# Autodesk Inventor assembly: wheel_kit
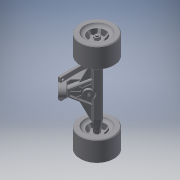
[picture p0: Inventor's stored thumbnail of the model, 180x180]
Saved by Autodesk Inventor 2017 SP1 (Build 210196100, 196)
## iProperties
Part Number: wheel_kit
Material: 一般
Document SubType Name: Assembly
Designer: gisen
Author: gisen
## Documents named in this file (5)
- C:\Users\gisen\Documents\myElectricSk8\CAD\wheel_kit.iam
- C:\Users\gisen\Documents\myElectricSk8\CAD\shaft.ipt
- C:\Users\gisen\Documents\myElectricSk8\CAD\wheel.ipt
- C:\Users\gisen\Documents\myElectricSk8\CAD\nut.ipt
- C:\Users\gisen\Documents\myElectricSk8\CAD\shaft_jig.ipt
## Components (6 placed, 4 different names)
1. shaft:1 — 円柱状:1, 円柱状:2, メイト:1, メイト:2, メイト:3, メイト:6, メイト:7, メイト:8, メイト:9, フラッシュ:1
2. wheel:1 — 円柱状:1, メイト:1, メイト:5
3. wheel:2 — 円柱状:2, メイト:2, メイト:4
4. nut:1 — メイト:3, メイト:4
5. nut:2 — メイト:5, メイト:6
6. shaft_jig:1 — メイト:7, メイト:8, メイト:9, メイト:10
## Relationships (13: Mate 10, CylindricalJoint 2, Flush 1)
- 円柱状:1 [CylindricalJoint]: shaft:1 ↔ wheel:1
- 円柱状:2 [CylindricalJoint]: shaft:1 ↔ wheel:2
- メイト:1 [Mate]: shaft:1 ↔ wheel:1
- メイト:2 [Mate]: shaft:1 ↔ wheel:2
- メイト:3 [Mate]: shaft:1 ↔ nut:1
- メイト:4 [Mate]: wheel:2 ↔ nut:1
- メイト:5 [Mate]: wheel:1 ↔ nut:2
- メイト:6 [Mate]: shaft:1 ↔ nut:2
- メイト:7 [Mate]: shaft:1 ↔ shaft_jig:1
- メイト:8 [Mate]: shaft:1 ↔ shaft_jig:1
- メイト:9 [Mate]: shaft:1 ↔ shaft_jig:1
- メイト:10 [Mate]: shaft_jig:1
- フラッシュ:1 [Flush]: shaft:1
